# Autodesk Inventor assembly: _WandAssembly
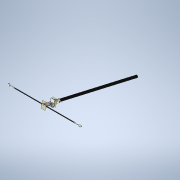
[picture p0: Inventor's stored thumbnail of the model, 180x180]
Saved by Autodesk Inventor 2022 (Build 260153000, 153)
## iProperties
Created: 2022-06-22
Part Number: _WandAssembly
Document SubType Name: Assembly
Designer: tecware
Author: tecware
## Documents named in this file (5)
- C:\Users\tecware\Documents\git\calibrationKit\calibrationKit_v2\wand\_WandAssembly.iam
- C:\Users\tecware\Documents\git\calibrationKit\calibrationKit_v2\wand\components_wand\horizontalRod.ipt
- C:\Users\tecware\Documents\git\calibrationKit\calibrationKit_v2\wand\components_wand\PVC_conduit.ipt
- C:\Users\tecware\Documents\git\calibrationKit\calibrationKit_v2\wand\components_wand\markerWithRodEnd_new1.ipt
- C:\Users\tecware\Documents\git\calibrationKit\calibrationKit_v2\wand\prototype_for_circuit&connections\prototype_11.iam
## Components (7 placed, 4 different names)
1. horizontalRod:1 — Mate:2, Mate:3, Rigid:1, Mate:10, Mate:11
2. PVC_conduit:1 — Mate:6, Mate:7
3. markerWithRodEnd_new1:1 — Mate:1, Flush:1, Mate:3, Mate:4
4. markerWithRodEnd_new1:2 — Mate:1, Flush:1, Mate:2, Mate:4
5. markerWithRodEnd_new1:3 — Mate:10, Mate:11
6. markerWithRodEnd_new1:4
7. prototype_11:1 [sub-assembly] — Mate:6, Mate:7, Rigid:1
## Relationships (13: Mate 10, Flush 2, WeldJoint 1)
- Mate:1: markerWithRodEnd_new1:1 ↔ markerWithRodEnd_new1:2
- Flush:1: markerWithRodEnd_new1:1 ↔ markerWithRodEnd_new1:2
- Mate:2: horizontalRod:1 ↔ markerWithRodEnd_new1:2
- Mate:3: horizontalRod:1 ↔ markerWithRodEnd_new1:1
- Mate:4: markerWithRodEnd_new1:1 ↔ markerWithRodEnd_new1:2
- Mate:6: PVC_conduit:1 ↔ prototype_11:1
- Mate:7: PVC_conduit:1 ↔ prototype_11:1
- Rigid:1 [WeldJoint]: horizontalRod:1 ↔ prototype_11:1
- [Mate]: markerWithRodEnd_new1:3 ↔ markerWithRodEnd_new1:4
- [Flush]: markerWithRodEnd_new1:3 ↔ markerWithRodEnd_new1:4
- [Mate]: markerWithRodEnd_new1:3 ↔ markerWithRodEnd_new1:4
- Mate:10: horizontalRod:1 ↔ markerWithRodEnd_new1:3
- Mate:11: horizontalRod:1 ↔ markerWithRodEnd_new1:3
## Named parameters: d17_d4 = 0 mm, d18_d5 = 0 mm, d19_d10 = 0 mm
